# Autodesk Inventor assembly: case
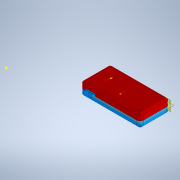
[picture p0: Inventor's stored thumbnail of the model, 180x180]
Saved by Autodesk Inventor 2020 (Build 240168000, 168)
## iProperties
Created: 2020-03-17
Part Number: case
Document SubType Name: Assembly
Designer: erwin
Author: erwin
## Documents named in this file (5)
- C:\Users\erwin\Documents\GitHub\pidflight-lap-firmware\case\v1_final\case.iam
- C:\Users\erwin\Documents\GitHub\pidflight-lap-firmware\case\v1_final\up.ipt
- C:\Users\erwin\Documents\GitHub\pidflight-lap-firmware\case\v1_final\down.ipt
- C:\Users\erwin\Documents\GitHub\pidflight-lap-firmware\case\v1_final\switch_slider.ipt
- C:\Users\erwin\Documents\GitHub\pidflight-lap-firmware\case\v1_final\switch_internal.ipt
## Components (4 placed, 4 different names)
1. up:1 — Mate:4, Flush:3, Flush:4
2. down:1 — Mate:2, Mate:3, Mate:4, Flush:3, Flush:4
3. switch_slider:1 — Mate:1, Mate:2, Mate:3, Flush:1, Flush:2
4. switch_internal:1 — Mate:1, Flush:1, Flush:2
## Relationships (8: Mate 4, Flush 4)
- Mate:1: switch_slider:1 ↔ switch_internal:1
- Mate:2 (0.5 mm): down:1 ↔ switch_slider:1
- Mate:3: down:1 ↔ switch_slider:1
- Flush:1 (3 mm): switch_slider:1 ↔ switch_internal:1
- Flush:2 (1 mm): switch_slider:1 ↔ switch_internal:1
- Mate:4: up:1 ↔ down:1
- Flush:3: up:1 ↔ down:1
- Flush:4: up:1 ↔ down:1
